# Autodesk Inventor assembly: OutputShaftAssembly
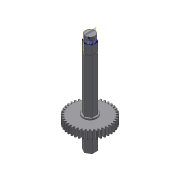
[picture p0: Inventor's stored thumbnail of the model, 180x180]
Saved by Autodesk Inventor 2013 SP1 (Build 170176100, 176)
## iProperties
Created: 2013-12-03
Part Number: OutputShaftAssembly
Document SubType Name: Assembly
Designer: robotics
Author: robotics
## Documents named in this file (3)
- C:\Users\robotics\Documents\GitHub\2014-Preseason-Single-Speed-Gearbox\manufacture\assemblies\OutputShaftAssembly.iam
- C:\Users\robotics\Documents\GitHub\2014-Preseason-Single-Speed-Gearbox\buy\VexPro\Gears\217-2708-STEP\Imported Components\217-2708.20121204\217-2708.20121204.ipt
- C:\Users\robotics\Documents\GitHub\2014-Preseason-Single-Speed-Gearbox\manufacture\parts\Shaft\OutputShaft.ipt
## Components (2 placed, 2 different names)
1. 217-2708.20121204:1 — Mate:1, Mate:2, Flush:1
2. OutputShaft:1 — Mate:1, Mate:2, Flush:1
## Relationships (3: Mate 2, Flush 1)
- Mate:1: 217-2708.20121204:1 ↔ OutputShaft:1
- Mate:2: 217-2708.20121204:1 ↔ OutputShaft:1
- Flush:1: 217-2708.20121204:1 ↔ OutputShaft:1
